# Autodesk Inventor assembly: full sincos
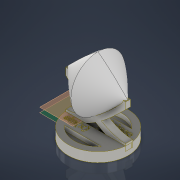
[picture p0: Inventor's stored thumbnail of the model, 180x180]
Saved by Autodesk Inventor 2022 (Build 260153000, 153)
## iProperties
Created: 2021-06-07
Part Number: full sincos
Document SubType Name: Assembly
Designer: sidsa
Author: sidsa
## Documents named in this file (4)
- D:\My Documents\gIThUB TWS\auto-dispenser\Inventor\3dp files\3d print test files\full sincos.iam
- D:\My Documents\gIThUB TWS\auto-dispenser\Inventor\3dp files\3d print test files\sincos half.ipt
- D:\My Documents\gIThUB TWS\auto-dispenser\Inventor\3dp files\3d print test files\sincos stand.ipt
- D:\My Documents\gIThUB TWS\auto-dispenser\Inventor\3dp files\3d print test files\sincos side display.ipt
## Components (4 placed, 3 different names)
1. sincos half:1 — Mate:2
2. sincos half:2 — Mate:2
3. sincos stand:1 — Mate:1
4. sincos side display:1 — Mate:1
## Relationships (2: Mate 2)
- Mate:1: sincos stand:1 ↔ sincos side display:1
- Mate:2: sincos half:1 ↔ sincos half:2
